# Autodesk Inventor assembly: 1254044 DHPS-16-A-NO---(10)
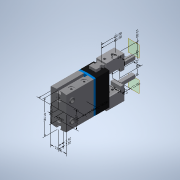
[picture p0: Inventor's stored thumbnail of the model, 180x180]
Saved by Autodesk Inventor 2020 (Build 240168000, 168)
## iProperties
Created: 2023-01-29
Part Number: 1254044 DHPS-16-A-NO---(10)
Catalog Web Link: www.cadenas.de
Description: DHPS-Parallel gripper
Vendor: FESTO
Document SubType Name: Assembly
Designer: psAdmin
Manufacturer: FESTO
Mass: 188 g
Surface Area: 194.692 cm^2
Volume: 62.4673 cm^3
Density: 3.00957 g/cm^3
Category: PARTsolutions
Company: FESTO
PSOL_IDENT_0: {ATYP=ASSISTANT},{DATA=script=$CADENAS_DATA/23d-libs/festo/webfesto.vbb/&M_FAMILY=DHPS&M_GROUP=01&M_
PSOL_IDENT_1: PARTNO=1254044&IDCODE1=DHPS-16-A-NO&IDCODE2=&customer_number_cns=&MATES=1&LOD=HI&LOCKERP=0&SINGLEPAR
PSOL_IDENT_2: T=1}
NB: 1254044 DHPS-16-A-NO---(10)
NN: DHPS
NT: Parallel gripper
NBSYN: $TNR. $TYP.---($HUBST.)
LINA: 1254044 DHPS-16-A-NO
CATALOG: Festo
TNR: 1254044
TYP: DHPS-16-A-NO
HUBST: 10
B1: 27.8
B2: 17.8
B3: 13
B4: 25
B5: 47
B6: 22.65
B7: 25
D1: 3
D2: 7
D3: 7
D4: 7
D5: 3.3
D6: M4
D7: 7
D8: 5.3
D9: M4
D10: 7
D11: 5.3
EE: M3
H1: 80
H2: 5.5
H3: 11
H4: 18
H5: 11
H6: 10
H7: 62.5
H8: 7.5
H9: 20
H10: 32.5
H11: 38.1
H12: 7
L1: 22
L2: 0
L3: 0
L4: 10
L5: 7
T1: 1.6
T2: 1.6
T3: 3
T4: 3
T5: 6
CNSMASSEXACT: 0.188
SUPPLIER: FESTO
ARTICLENO: 1254044 DHPS-16-A-NO---(10)
BOMINFO: 1254044 DHPS-16-A-NO
CREATOR: CADENAS GmbH
Title: 1254044 DHPS-16-A-NO
Author: Cadenas PARTsolutions
Comments: Parallel gripper
## Documents named in this file (5)
- C:\Users\ma203\Desktop\AIS2020\1254044 DHPS-16-A-NO---(10).iam
- C:\Users\ma203\Desktop\AIS2020\1254044 DHPS-16-A-NO---(Geh).ipt
- C:\Users\ma203\Desktop\AIS2020\186717 ZBH-7.ipt
- C:\Users\ma203\Desktop\AIS2020\1254044 DHPS-16-A-NO---(Handle).ipt
- C:\Users\ma203\Desktop\AIS2020\Part2.ipt
## Components (9 placed, 4 different names)
1. 1254044 DHPS-16-A-NO---(Geh):1 — TO_ZBH_1_Z@1 <-> insert_Z@2, TO_ZBH_1_YZ@1 <-> insert_YZ@2, TO_ZBH_2_Z@1 <-> insert_Z@3, TO_ZBH_2_YZ@1 <-> insert_YZ@3, TO_GREIF_XY@1 <-> GRIFF_XY@4, TO_GREIF_Z@1 <-> GRIFF_Z@4, TO_GREIF_YZ@1 <-> GRIFF_YZ@4, TO_GREIF_R_XY@1 <-> GRIFF_XY@7, TO_GREIF_R_Z@1 <-> GRIFF_Z@7, TO_GREIF_R_YZ@1 <-> GRIFF_YZ@7
2. 186717 ZBH-7:1 — TO_ZBH_1_Z@1 <-> insert_Z@2, TO_ZBH_1_YZ@1 <-> insert_YZ@2
3. 186717 ZBH-7:2 — TO_ZBH_2_Z@1 <-> insert_Z@3, TO_ZBH_2_YZ@1 <-> insert_YZ@3
4. 1254044 DHPS-16-A-NO---(Handle):1 — TO_GREIF_XY@1 <-> GRIFF_XY@4, TO_GREIF_Z@1 <-> GRIFF_Z@4, TO_GREIF_YZ@1 <-> GRIFF_YZ@4, Mate:18, Mate:19, Mate:20
5. 1254044 DHPS-16-A-NO---(Handle):2 — TO_GREIF_R_XY@1 <-> GRIFF_XY@7, TO_GREIF_R_Z@1 <-> GRIFF_Z@7, TO_GREIF_R_YZ@1 <-> GRIFF_YZ@7, TO_ZBH_1_XY@7 <-> insert_XY@8, TO_ZBH_1_Z@7 <-> insert_Z@8, TO_ZBH_1_YZ@7 <-> insert_YZ@8, TO_ZBH_2_XY@7 <-> insert_XY@9, TO_ZBH_2_Z@7 <-> insert_Z@9, TO_ZBH_2_YZ@7 <-> insert_YZ@9, Mate:15, Mate:16, Mate:17
6. 186717 ZBH-7:5 — TO_ZBH_1_XY@7 <-> insert_XY@8, TO_ZBH_1_Z@7 <-> insert_Z@8, TO_ZBH_1_YZ@7 <-> insert_YZ@8
7. 186717 ZBH-7:6 — TO_ZBH_2_XY@7 <-> insert_XY@9, TO_ZBH_2_Z@7 <-> insert_Z@9, TO_ZBH_2_YZ@7 <-> insert_YZ@9
8. Part2:1 — Mate:15, Mate:16, Mate:17
9. Part2:2 — Mate:18, Mate:19, Mate:20
## Relationships (22: Mate 16, Angle 6)
- TO_ZBH_1_Z@1 <-> insert_Z@2 [Mate]: 1254044 DHPS-16-A-NO---(Geh):1 ↔ 186717 ZBH-7:1
- TO_ZBH_1_YZ@1 <-> insert_YZ@2 [Angle] (0 deg): 1254044 DHPS-16-A-NO---(Geh):1 ↔ 186717 ZBH-7:1
- TO_ZBH_2_Z@1 <-> insert_Z@3 [Mate]: 1254044 DHPS-16-A-NO---(Geh):1 ↔ 186717 ZBH-7:2
- TO_ZBH_2_YZ@1 <-> insert_YZ@3 [Angle] (0 deg): 1254044 DHPS-16-A-NO---(Geh):1 ↔ 186717 ZBH-7:2
- TO_GREIF_XY@1 <-> GRIFF_XY@4 [Mate] (5 mm): 1254044 DHPS-16-A-NO---(Geh):1 ↔ 1254044 DHPS-16-A-NO---(Handle):1
- TO_GREIF_Z@1 <-> GRIFF_Z@4 [Mate]: 1254044 DHPS-16-A-NO---(Geh):1 ↔ 1254044 DHPS-16-A-NO---(Handle):1
- TO_GREIF_YZ@1 <-> GRIFF_YZ@4 [Angle] (0 deg): 1254044 DHPS-16-A-NO---(Geh):1 ↔ 1254044 DHPS-16-A-NO---(Handle):1
- TO_GREIF_R_XY@1 <-> GRIFF_XY@7 [Mate] (5 mm): 1254044 DHPS-16-A-NO---(Geh):1 ↔ 1254044 DHPS-16-A-NO---(Handle):2
- TO_GREIF_R_Z@1 <-> GRIFF_Z@7 [Mate]: 1254044 DHPS-16-A-NO---(Geh):1 ↔ 1254044 DHPS-16-A-NO---(Handle):2
- TO_GREIF_R_YZ@1 <-> GRIFF_YZ@7 [Angle] (0 deg): 1254044 DHPS-16-A-NO---(Geh):1 ↔ 1254044 DHPS-16-A-NO---(Handle):2
- TO_ZBH_1_XY@7 <-> insert_XY@8 [Mate]: 1254044 DHPS-16-A-NO---(Handle):2 ↔ 186717 ZBH-7:5
- TO_ZBH_1_Z@7 <-> insert_Z@8 [Mate]: 1254044 DHPS-16-A-NO---(Handle):2 ↔ 186717 ZBH-7:5
- TO_ZBH_1_YZ@7 <-> insert_YZ@8 [Angle] (0 deg): 1254044 DHPS-16-A-NO---(Handle):2 ↔ 186717 ZBH-7:5
- TO_ZBH_2_XY@7 <-> insert_XY@9 [Mate]: 1254044 DHPS-16-A-NO---(Handle):2 ↔ 186717 ZBH-7:6
- TO_ZBH_2_Z@7 <-> insert_Z@9 [Mate]: 1254044 DHPS-16-A-NO---(Handle):2 ↔ 186717 ZBH-7:6
- TO_ZBH_2_YZ@7 <-> insert_YZ@9 [Angle] (0 deg): 1254044 DHPS-16-A-NO---(Handle):2 ↔ 186717 ZBH-7:6
- Mate:15: 1254044 DHPS-16-A-NO---(Handle):2 ↔ Part2:1
- Mate:16: 1254044 DHPS-16-A-NO---(Handle):2 ↔ Part2:1
- Mate:17: 1254044 DHPS-16-A-NO---(Handle):2 ↔ Part2:1
- Mate:18: 1254044 DHPS-16-A-NO---(Handle):1 ↔ Part2:2
- Mate:19: 1254044 DHPS-16-A-NO---(Handle):1 ↔ Part2:2
- Mate:20: 1254044 DHPS-16-A-NO---(Handle):1 ↔ Part2:2
